# Autodesk Inventor assembly: Assembly1
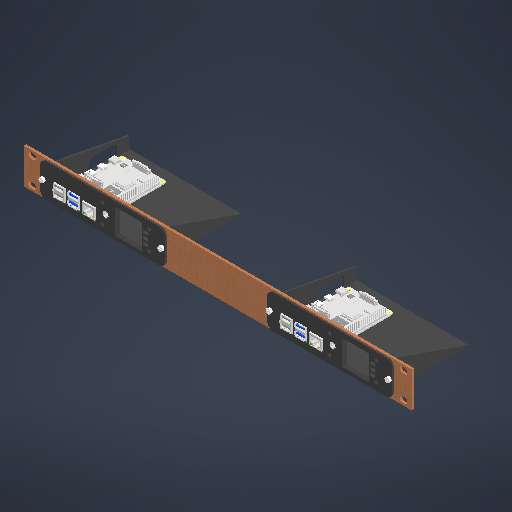
[picture p0: Inventor's stored thumbnail of the model, 512x512]
Saved by Autodesk Inventor 2026.2 (Build 302298010, 298A)
## iProperties
Created: 2026-03-25
Part Number: Assembly1
Document SubType Name: Assembly
Designer: usr
Author: usr
## Documents named in this file (5)
- C:\Users\usr\Documents\GitHub\2526-ITF-003-ip-terminals-netwerklokalen\3d\Assembly1.iam
- C:\Users\usr\Documents\GitHub\2526-ITF-003-ip-terminals-netwerklokalen\3d\WoodPanel.ipt
- C:\Users\usr\Documents\GitHub\2526-ITF-003-ip-terminals-netwerklokalen\3d\M3 hex nut v6.ipt
- C:\Users\usr\Documents\GitHub\2526-ITF-003-ip-terminals-netwerklokalen\3d\BoltM3-PI-2.ipt
- C:\Users\usr\Documents\GitHub\2526-ITF-003-ip-terminals-netwerklokalen\3d\PI-RACK-MOUNT.iam
## Components (11 placed, 4 different names)
1. WoodPanel:1 — Mate:40, Mate:41, Mate:42, Mate:47, Mate:49, Mate:51, Mate:52
2. M3 hex nut v6:4 — Mate:47, Mate:48
3. M3 hex nut v6:5 — Mate:49, Mate:50
4. PI-RACK-MOUNT:2 [sub-assembly] — Mate:40, Mate:41, Mate:42, Mate:44, Mate:46
5. PI-RACK-MOUNT:1 [sub-assembly] — Mate:36, Mate:37, Mate:38, Mate:39
6. BoltM3-PI-2:6 — Mate:46, Mate:48, Mate:52
7. BoltM3-PI-2:5 — Mate:44, Mate:50, Mate:51
8. BoltM3-PI-2:3 — Mate:36, Mate:39
9. BoltM3-PI-2:4 — Mate:37, Mate:38
10. M3 hex nut v6:2
11. M3 hex nut v6:3
## Relationships (18: Mate 18)
- [Mate]: WoodPanel:1 ↔ PI-RACK-MOUNT:1
- [Mate]: WoodPanel:1 ↔ PI-RACK-MOUNT:1
- [Mate]: WoodPanel:1 ↔ PI-RACK-MOUNT:1
- Mate:36: PI-RACK-MOUNT:1 ↔ BoltM3-PI-2:3
- Mate:37: PI-RACK-MOUNT:1 ↔ BoltM3-PI-2:4
- Mate:38: PI-RACK-MOUNT:1 ↔ BoltM3-PI-2:4
- Mate:39: PI-RACK-MOUNT:1 ↔ BoltM3-PI-2:3
- Mate:40: WoodPanel:1 ↔ PI-RACK-MOUNT:2
- Mate:41: WoodPanel:1 ↔ PI-RACK-MOUNT:2
- Mate:42: WoodPanel:1 ↔ PI-RACK-MOUNT:2
- Mate:44: PI-RACK-MOUNT:2 ↔ BoltM3-PI-2:5
- Mate:46: PI-RACK-MOUNT:2 ↔ BoltM3-PI-2:6
- Mate:47: WoodPanel:1 ↔ M3 hex nut v6:4
- Mate:48: M3 hex nut v6:4 ↔ BoltM3-PI-2:6
- Mate:49: WoodPanel:1 ↔ M3 hex nut v6:5
- Mate:50: M3 hex nut v6:5 ↔ BoltM3-PI-2:5
- Mate:51: WoodPanel:1 ↔ BoltM3-PI-2:5
- Mate:52: WoodPanel:1 ↔ BoltM3-PI-2:6
